# Autodesk Inventor assembly: side of drivetrain
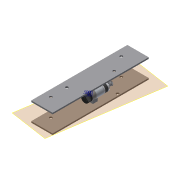
[picture p0: Inventor's stored thumbnail of the model, 180x180]
Saved by Autodesk Inventor 2020 (Build 240168000, 168)
## iProperties
Created: 2019-10-04
Part Number: side of drivetrain
Document SubType Name: Assembly
Designer: ball
Author: ball
## Documents named in this file (6)
- C:\FTC\FTC8863CAD\2019 Robot\Mecanum Drive Train\side of drivetrain gb.iam
- C:\FTC\FTC8863CAD\2019 Robot\Mecanum Drive Train\wheel with drive motor top.iam
- C:\FTC\FTC8863CAD\2019 Robot\Mecanum Drive Train\wheel with drive motor floor.iam
- C:\FTC\FTC8863CAD\2019 Robot\Mecanum Drive Train\inside wall.ipt
- C:\FTC\FTC8863CAD\2019 Robot\Mecanum Drive Train\outside wall.ipt
- C:\FTC\FTC8863CAD\2019 Robot\Mecanum Drive Train\center motor mount.ipt
## Components (5 placed, 5 different names)
1. wheel with drive motor top:1 [sub-assembly] — Flush:4, Mate:3, Mate:5, Flush:6, Mate:6, Mate:7, Mate:8
2. wheel with drive motor floor:1 [sub-assembly] — Flush:4, Mate:4, Mate:5, Flush:6, Mate:9
3. outside wall:1 — Mate:3, Mate:4, Mate:6, Mate:10, Flush:7, Flush:8
4. inside wall — Mate:7, Mate:8, Mate:9, Mate:11
5. center motor mount:1 — Flush:7, Flush:8
## Relationships (13: Mate 9, Flush 4)
- Flush:4: wheel with drive motor top:1 ↔ wheel with drive motor floor:1
- Mate:3: wheel with drive motor top:1 ↔ outside wall:1
- Mate:4: wheel with drive motor floor:1 ↔ outside wall:1
- Mate:5 (44.3484 mm): wheel with drive motor top:1 ↔ wheel with drive motor floor:1
- Flush:6 (330.2 mm): wheel with drive motor top:1 ↔ wheel with drive motor floor:1
- Mate:6: wheel with drive motor top:1 ↔ outside wall:1
- Mate:7: wheel with drive motor top:1 ↔ inside wall
- Mate:8: wheel with drive motor top:1 ↔ inside wall
- Mate:9: wheel with drive motor floor:1 ↔ inside wall
- Mate:10: outside wall:1
- Mate:11: inside wall
- Flush:7: outside wall:1 ↔ center motor mount:1
- Flush:8: outside wall:1 ↔ center motor mount:1
